# Autodesk Inventor assembly: Rocket
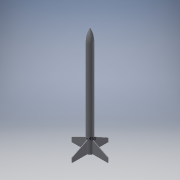
[picture p0: Inventor's stored thumbnail of the model, 180x180]
Saved by Autodesk Inventor 2016 (Build 200138000, 138)
## iProperties
Created: 2015-06-24
Part Number: Rocket
Document SubType Name: Assembly
Designer: The Shack
Author: The Shack
## Documents named in this file (4)
- C:\Users\The Shack\Dropbox\Andrew\Rocket.iam
- C:\Users\The Shack\Dropbox\Andrew\Rocket - Base Assembled.ipt
- C:\Users\The Shack\Dropbox\Andrew\Rocket - Shaft.ipt
- C:\Users\The Shack\Dropbox\Andrew\Rocket - Nose Cone.ipt
## Components (3 placed, 3 different names)
1. Rocket - Base Assembled:1 — Mate:1
2. Rocket - Shaft:1 — Insert:1, Mate:1
3. Rocket - Nose Cone:1 — Insert:1
## Relationships (2: Insert 1, Mate 1)
- Insert:1: Rocket - Shaft:1 ↔ Rocket - Nose Cone:1
- Mate:1: Rocket - Base Assembled:1 ↔ Rocket - Shaft:1
